# Autodesk Inventor assembly: zespół płyty
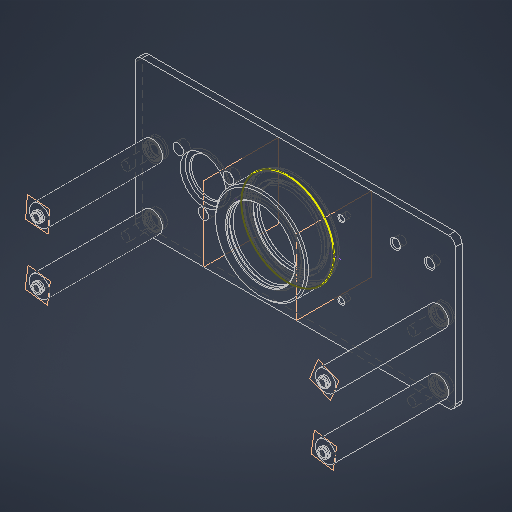
[picture p0: Inventor's stored thumbnail of the model, 512x512]
Saved by Autodesk Inventor 2026.1 (Build 301233020, 233B)
## iProperties
Created: 2026-04-19
Part Number: zespół płyty
Document SubType Name: Assembly
Designer: Jan
Author: Jan
## Documents named in this file (4)
- C:\Users\Jan\OneDrive\Pulpit\Ainventor-ZNL\czesci\zespół płyty.iam
- C:\Users\Jan\OneDrive\Pulpit\Ainventor-ZNL\czesci\płyta silnika.ipt
- C:\Users\Jan\OneDrive\Pulpit\Ainventor-ZNL\czesci\słupek.ipt
- C:\Users\Jan\OneDrive\Pulpit\Ainventor-ZNL\czesci\tuleja łożyska.ipt
## Components (6 placed, 3 different names)
1. płyta silnika:1 — Mate:1, Mate:2, Mate:3, Mate:4, Mate:5, Mate:6, Mate:7, Mate:8, Mate:9, Mate:10
2. słupek:1 — Mate:1, Mate:8
3. słupek:2 — Mate:2, Mate:7
4. słupek:3 — Mate:3, Mate:10
5. słupek:4 — Mate:4, Mate:9
6. tuleja łożyska:1 — Mate:5, Mate:6
## Relationships (10: Mate 10)
- Mate:1: płyta silnika:1 ↔ słupek:1
- Mate:2: płyta silnika:1 ↔ słupek:2
- Mate:3: płyta silnika:1 ↔ słupek:3
- Mate:4: płyta silnika:1 ↔ słupek:4
- Mate:5: płyta silnika:1 ↔ tuleja łożyska:1
- Mate:6: płyta silnika:1 ↔ tuleja łożyska:1
- Mate:7: płyta silnika:1 ↔ słupek:2
- Mate:8: płyta silnika:1 ↔ słupek:1
- Mate:9: płyta silnika:1 ↔ słupek:4
- Mate:10: płyta silnika:1 ↔ słupek:3
